# Autodesk Inventor assembly: Sliding Elevator Block Assembly <1>
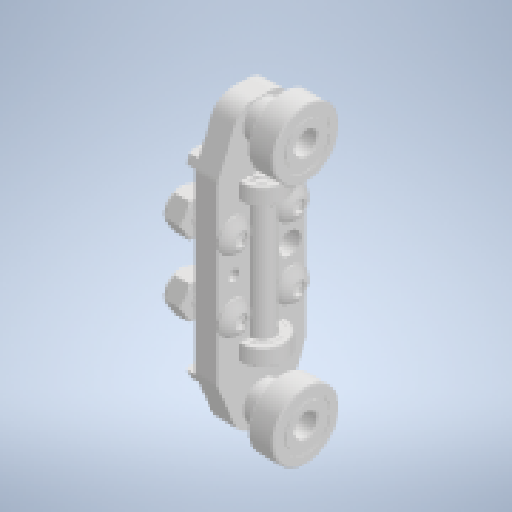
[picture p0: Inventor's stored thumbnail of the model, 512x512]
Saved by Autodesk Inventor 2023 (Build 270158000, 158)
## iProperties
Created: 2023-01-16
Part Number: Sliding Elevator Block Assembly <1>
Description: Sliding Elevator Block Assembly <1>
Document SubType Name: Assembly
Designer: Gabriel - T3 CAD
Author: Gabriel - T3 CAD
## Documents named in this file (54)
- C:\Users\Gabriel - T3 CAD\Documents\GitHub\t3-CAD\T3-CAD\Stock\ThriftyBot-Elevator\New folder\Sliding Elevator Block Assembly _1_.iam
- C:\Users\Gabriel - T3 CAD\Documents\GitHub\t3-CAD\T3-CAD\Stock\ThriftyBot-Elevator\New folder\Bearing Block Shoulder Bolt Spacer - SLIDE-003_1.ipt
- C:\Users\Gabriel - T3 CAD\Documents\GitHub\t3-CAD\T3-CAD\Stock\ThriftyBot-Elevator\New folder\10-32 Locknut 2623_2_1.ipt
- C:\Users\Gabriel - T3 CAD\Documents\GitHub\t3-CAD\T3-CAD\Stock\ThriftyBot-Elevator\New folder\TTB-0027_.50OD_.25ID_.188WD_15.ipt
- C:\Users\Gabriel - T3 CAD\Documents\GitHub\t3-CAD\T3-CAD\Stock\ThriftyBot-Elevator\New folder\Bearing Block Shoulder Bolt Spacer - SLIDE-003.ipt
- C:\Users\Gabriel - T3 CAD\Documents\GitHub\t3-CAD\T3-CAD\Stock\ThriftyBot-Elevator\New folder\TTB-0027_.50OD_.25ID_.188WD_1_6.ipt
- C:\Users\Gabriel - T3 CAD\Documents\GitHub\t3-CAD\T3-CAD\Stock\ThriftyBot-Elevator\New folder\TTB-0027_.50OD_.25ID_.188WD_1.ipt
- C:\Users\Gabriel - T3 CAD\Documents\GitHub\t3-CAD\T3-CAD\Stock\ThriftyBot-Elevator\New folder\TTB-0027_.50OD_.25ID_.188WD_6.ipt
- C:\Users\Gabriel - T3 CAD\Documents\GitHub\t3-CAD\T3-CAD\Stock\ThriftyBot-Elevator\New folder\.625 Long 10-32 Button Head Screw 13116.ipt
- C:\Users\Gabriel - T3 CAD\Documents\GitHub\t3-CAD\T3-CAD\Stock\ThriftyBot-Elevator\New folder\TTB-0027_.50OD_.25ID_.188WD_10.ipt
- C:\Users\Gabriel - T3 CAD\Documents\GitHub\t3-CAD\T3-CAD\Stock\ThriftyBot-Elevator\New folder\.25diameter_1.75inSteelDowel_SLIDE-002.ipt
- C:\Users\Gabriel - T3 CAD\Documents\GitHub\t3-CAD\T3-CAD\Stock\ThriftyBot-Elevator\New folder\TTB-0027_.50OD_.25ID_.188WD_1_5.ipt
- C:\Users\Gabriel - T3 CAD\Documents\GitHub\t3-CAD\T3-CAD\Stock\ThriftyBot-Elevator\New folder\10-32 Locknut 2623_1.ipt
- C:\Users\Gabriel - T3 CAD\Documents\GitHub\t3-CAD\T3-CAD\Stock\ThriftyBot-Elevator\New folder\TTB-0027_.50OD_.25ID_.188WD_12.ipt
- C:\Users\Gabriel - T3 CAD\Documents\GitHub\t3-CAD\T3-CAD\Stock\ThriftyBot-Elevator\New folder\TTB-0027_.50OD_.25ID_.188WD_1_13.ipt
- C:\Users\Gabriel - T3 CAD\Documents\GitHub\t3-CAD\T3-CAD\Stock\ThriftyBot-Elevator\New folder\TTB-0027_.50OD_.25ID_.188WD_1_1.ipt
- C:\Users\Gabriel - T3 CAD\Documents\GitHub\t3-CAD\T3-CAD\Stock\ThriftyBot-Elevator\New folder\TTB-0027_.50OD_.25ID_.188WD_1_2.ipt
- C:\Users\Gabriel - T3 CAD\Documents\GitHub\t3-CAD\T3-CAD\Stock\ThriftyBot-Elevator\New folder\TTB-0027_.50OD_.25ID_.188WD_14.ipt
- C:\Users\Gabriel - T3 CAD\Documents\GitHub\t3-CAD\T3-CAD\Stock\ThriftyBot-Elevator\New folder\TTB-0027_.50OD_.25ID_.188WD_7.ipt
- C:\Users\Gabriel - T3 CAD\Documents\GitHub\t3-CAD\T3-CAD\Stock\ThriftyBot-Elevator\New folder\10-32 Locknut 2623_2.ipt
- C:\Users\Gabriel - T3 CAD\Documents\GitHub\t3-CAD\T3-CAD\Stock\ThriftyBot-Elevator\New folder\Sliding Bearing Block Plate - SLIDE-001.ipt
- C:\Users\Gabriel - T3 CAD\Documents\GitHub\t3-CAD\T3-CAD\Stock\ThriftyBot-Elevator\New folder\.625 Long 10-32 Button Head Screw 13116_3.ipt
- C:\Users\Gabriel - T3 CAD\Documents\GitHub\t3-CAD\T3-CAD\Stock\ThriftyBot-Elevator\New folder\10-32 Locknut 2623_3_1.ipt
- C:\Users\Gabriel - T3 CAD\Documents\GitHub\t3-CAD\T3-CAD\Stock\ThriftyBot-Elevator\New folder\10-32 Locknut 2623.ipt
- C:\Users\Gabriel - T3 CAD\Documents\GitHub\t3-CAD\T3-CAD\Stock\ThriftyBot-Elevator\New folder\10-32 Locknut 2623_4.ipt
- C:\Users\Gabriel - T3 CAD\Documents\GitHub\t3-CAD\T3-CAD\Stock\ThriftyBot-Elevator\New folder\TTB-0027_.50OD_.25ID_.188WD_5.ipt
- C:\Users\Gabriel - T3 CAD\Documents\GitHub\t3-CAD\T3-CAD\Stock\ThriftyBot-Elevator\New folder\TTB-0027_.50OD_.25ID_.188WD_1_7.ipt
- C:\Users\Gabriel - T3 CAD\Documents\GitHub\t3-CAD\T3-CAD\Stock\ThriftyBot-Elevator\New folder\TTB-0027_.50OD_.25ID_.188WD_1_10.ipt
- C:\Users\Gabriel - T3 CAD\Documents\GitHub\t3-CAD\T3-CAD\Stock\ThriftyBot-Elevator\New folder\TTB-0027_.50OD_.25ID_.188WD_11.ipt
- C:\Users\Gabriel - T3 CAD\Documents\GitHub\t3-CAD\T3-CAD\Stock\ThriftyBot-Elevator\New folder\TTB-0038_75OD_25ID_28WD_1_1.ipt
- C:\Users\Gabriel - T3 CAD\Documents\GitHub\t3-CAD\T3-CAD\Stock\ThriftyBot-Elevator\New folder\TTB-0027_.50OD_.25ID_.188WD.ipt
- C:\Users\Gabriel - T3 CAD\Documents\GitHub\t3-CAD\T3-CAD\Stock\ThriftyBot-Elevator\New folder\TTB-0027_.50OD_.25ID_.188WD_9.ipt
- C:\Users\Gabriel - T3 CAD\Documents\GitHub\t3-CAD\T3-CAD\Stock\ThriftyBot-Elevator\New folder\TTB-0027_.50OD_.25ID_.188WD_8.ipt
- C:\Users\Gabriel - T3 CAD\Documents\GitHub\t3-CAD\T3-CAD\Stock\ThriftyBot-Elevator\New folder\TTB-0027_.50OD_.25ID_.188WD_4.ipt
- C:\Users\Gabriel - T3 CAD\Documents\GitHub\t3-CAD\T3-CAD\Stock\ThriftyBot-Elevator\New folder\TTB-0027_.50OD_.25ID_.188WD_3.ipt
- C:\Users\Gabriel - T3 CAD\Documents\GitHub\t3-CAD\T3-CAD\Stock\ThriftyBot-Elevator\New folder\TTB-0038_75OD_25ID_28WD_1_2.ipt
- C:\Users\Gabriel - T3 CAD\Documents\GitHub\t3-CAD\T3-CAD\Stock\ThriftyBot-Elevator\New folder\10-32 Locknut 2623_1_1.ipt
- C:\Users\Gabriel - T3 CAD\Documents\GitHub\t3-CAD\T3-CAD\Stock\ThriftyBot-Elevator\New folder\TTB-0027_.50OD_.25ID_.188WD_16.ipt
- C:\Users\Gabriel - T3 CAD\Documents\GitHub\t3-CAD\T3-CAD\Stock\ThriftyBot-Elevator\New folder\TTB-0027_.50OD_.25ID_.188WD_1_11.ipt
- C:\Users\Gabriel - T3 CAD\Documents\GitHub\t3-CAD\T3-CAD\Stock\ThriftyBot-Elevator\New folder\.625 Long 10-32 Button Head Screw 13116_2.ipt
- C:\Users\Gabriel - T3 CAD\Documents\GitHub\t3-CAD\T3-CAD\Stock\ThriftyBot-Elevator\New folder\TTB-0027_.50OD_.25ID_.188WD_1_8.ipt
- C:\Users\Gabriel - T3 CAD\Documents\GitHub\t3-CAD\T3-CAD\Stock\ThriftyBot-Elevator\New folder\TTB-0038_75OD_25ID_28WD_1.ipt
- C:\Users\Gabriel - T3 CAD\Documents\GitHub\t3-CAD\T3-CAD\Stock\ThriftyBot-Elevator\New folder\.625 Long 10-32 Button Head Screw 13116_1.ipt
- C:\Users\Gabriel - T3 CAD\Documents\GitHub\t3-CAD\T3-CAD\Stock\ThriftyBot-Elevator\New folder\10-32 Locknut 2623_3.ipt
- C:\Users\Gabriel - T3 CAD\Documents\GitHub\t3-CAD\T3-CAD\Stock\ThriftyBot-Elevator\New folder\TTB-0027_.50OD_.25ID_.188WD_1_4.ipt
- C:\Users\Gabriel - T3 CAD\Documents\GitHub\t3-CAD\T3-CAD\Stock\ThriftyBot-Elevator\New folder\TTB-0038_75OD_25ID_28WD.ipt
- C:\Users\Gabriel - T3 CAD\Documents\GitHub\t3-CAD\T3-CAD\Stock\ThriftyBot-Elevator\New folder\TTB-0027_.50OD_.25ID_.188WD_1_3.ipt
- C:\Users\Gabriel - T3 CAD\Documents\GitHub\t3-CAD\T3-CAD\Stock\ThriftyBot-Elevator\New folder\TTB-0027_.50OD_.25ID_.188WD_13.ipt
- C:\Users\Gabriel - T3 CAD\Documents\GitHub\t3-CAD\T3-CAD\Stock\ThriftyBot-Elevator\New folder\TTB-0027_.50OD_.25ID_.188WD_1_14.ipt
- C:\Users\Gabriel - T3 CAD\Documents\GitHub\t3-CAD\T3-CAD\Stock\ThriftyBot-Elevator\New folder\TTB-0027_.50OD_.25ID_.188WD_1_12.ipt
- C:\Users\Gabriel - T3 CAD\Documents\GitHub\t3-CAD\T3-CAD\Stock\ThriftyBot-Elevator\New folder\TTB-0027_.50OD_.25ID_.188WD_1_15.ipt
- C:\Users\Gabriel - T3 CAD\Documents\GitHub\t3-CAD\T3-CAD\Stock\ThriftyBot-Elevator\New folder\TTB-0027_.50OD_.25ID_.188WD_2.ipt
- C:\Users\Gabriel - T3 CAD\Documents\GitHub\t3-CAD\T3-CAD\Stock\ThriftyBot-Elevator\New folder\TTB-0027_.50OD_.25ID_.188WD_1_9.ipt
- C:\Users\Gabriel - T3 CAD\Documents\GitHub\t3-CAD\T3-CAD\Stock\Fasteners\91259A102_NO THREADS_Alloy Steel Shoulder Screw.ipt
## Components (54 placed, 53 different names)
1. NAUO210
2. NAUO211
3. NAUO212
4. NAUO213
5. NAUO214
6. NAUO215
7. NAUO217
8. NAUO218
9. NAUO219
10. NAUO220
11. NAUO221
12. NAUO222
13. NAUO223
14. NAUO224
15. NAUO225
16. NAUO226
17. NAUO227
18. NAUO228
19. NAUO229
20. NAUO230 — Mate:1, Mate:2, Mate:3, Mate:4
21. NAUO231
22. NAUO232
23. NAUO233
24. NAUO234
25. NAUO235
26. NAUO236
27. NAUO237
28. NAUO238
29. NAUO239
30. NAUO240
31. NAUO241
32. NAUO242
33. NAUO243
34. NAUO244
35. NAUO245
36. NAUO246
37. NAUO247
38. NAUO248
39. NAUO249
40. NAUO250
41. NAUO251
42. NAUO252
43. NAUO253
44. NAUO254
45. NAUO255
46. NAUO256
47. NAUO257
48. NAUO258
49. NAUO259
50. NAUO261
51. NAUO262
52. NAUO263
53. 91259A102_NO THREADS_Alloy Steel Shoulder Screw:1 — Mate:2, Mate:3
54. 91259A102_NO THREADS_Alloy Steel Shoulder Screw:2 — Mate:1, Mate:4
## Relationships (4: Mate 4)
- Mate:1: NAUO230 ↔ 91259A102_NO THREADS_Alloy Steel Shoulder Screw:2
- Mate:2: NAUO230 ↔ 91259A102_NO THREADS_Alloy Steel Shoulder Screw:1
- Mate:3: NAUO230 ↔ 91259A102_NO THREADS_Alloy Steel Shoulder Screw:1
- Mate:4: NAUO230 ↔ 91259A102_NO THREADS_Alloy Steel Shoulder Screw:2
